# Autodesk Inventor assembly: Gaveta
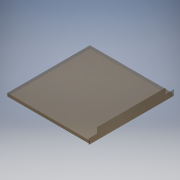
[picture p0: Inventor's stored thumbnail of the model, 180x180]
Saved by Autodesk Inventor 2018 (Build 220112000, 112)
## iProperties
Created: 2018-07-08
Part Number: Gaveta
Material: Genérico
Document SubType Name: Assembly
Designer: Regner
Author: Regner
## Documents named in this file (5)
- C:\Users\Regner\Documents\ROBOTA\2018\Tortura Ratos\Gaveta.iam
- C:\Users\Regner\Documents\ROBOTA\2018\Tortura Ratos\Tampa Gaveta.ipt
- C:\Users\Regner\Documents\ROBOTA\2018\Tortura Ratos\Fundo Gaveta.ipt
- C:\Users\Regner\Documents\ROBOTA\2018\Tortura Ratos\Lateral 1 Gaveta.ipt
- C:\Users\Regner\Documents\ROBOTA\2018\Tortura Ratos\Lateral 2 Gaveta.ipt
## Components (5 placed, 4 different names)
1. Tampa Gaveta:1 — Coincidência:1, Alinhamento:1, Alinhamento:2, Coincidência:5, Coincidência:6
2. Fundo Gaveta:1 — Coincidência:1, Alinhamento:1, Alinhamento:2, Coincidência:2, Alinhamento:3, Alinhamento:4, Coincidência:3, Coincidência:4, Alinhamento:5, Alinhamento:6
3. Lateral 1 Gaveta:1 — Coincidência:2, Alinhamento:3, Alinhamento:4
4. Lateral 2 Gaveta:1 — Coincidência:4, Coincidência:5, Alinhamento:5
5. Lateral 2 Gaveta:2 — Coincidência:3, Coincidência:6, Alinhamento:6
## Relationships (12: Mate 6, Flush 6)
- Coincidência:1 [Mate]: Tampa Gaveta:1 ↔ Fundo Gaveta:1
- Alinhamento:1 [Flush]: Tampa Gaveta:1 ↔ Fundo Gaveta:1
- Alinhamento:2 [Flush] (4.4 mm): Tampa Gaveta:1 ↔ Fundo Gaveta:1
- Coincidência:2 [Mate]: Fundo Gaveta:1 ↔ Lateral 1 Gaveta:1
- Alinhamento:3 [Flush]: Fundo Gaveta:1 ↔ Lateral 1 Gaveta:1
- Alinhamento:4 [Flush]: Fundo Gaveta:1 ↔ Lateral 1 Gaveta:1
- Coincidência:3 [Mate]: Fundo Gaveta:1 ↔ Lateral 2 Gaveta:2
- Coincidência:4 [Mate]: Fundo Gaveta:1 ↔ Lateral 2 Gaveta:1
- Coincidência:5 [Mate]: Tampa Gaveta:1 ↔ Lateral 2 Gaveta:1
- Coincidência:6 [Mate]: Tampa Gaveta:1 ↔ Lateral 2 Gaveta:2
- Alinhamento:5 [Flush]: Fundo Gaveta:1 ↔ Lateral 2 Gaveta:1
- Alinhamento:6 [Flush]: Fundo Gaveta:1 ↔ Lateral 2 Gaveta:2
